# Autodesk Inventor assembly: TR2 Arm
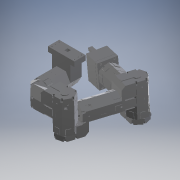
[picture p0: Inventor's stored thumbnail of the model, 180x180]
Saved by Autodesk Inventor 2017 (Build 210142000, 142)
## iProperties
Created: 2018-10-11
Part Number: TR2 Arm
Document SubType Name: Assembly
Designer: Zach
Author: Zach
## Documents named in this file (10)
- C:\Users\Dell\Documents\GitHub\tr2\Arm\Arm.iam
- C:\Users\Dell\Documents\GitHub\tr2\Arm Actuator\Arm Actuator.iam
- C:\Users\Dell\Documents\GitHub\tr2\Gripper\Gripper.iam
- C:\Users\Dell\Documents\GitHub\tr2\Arm\TARM04b.ipt
- C:\Users\Dell\Documents\GitHub\tr2\Arm\TARM09b.ipt
- C:\Users\Dell\Documents\GitHub\tr2\Arm\TARM01b.ipt
- C:\Users\Dell\Documents\GitHub\tr2\Arm\TARM02b.ipt
- C:\Users\Dell\Documents\GitHub\tr2\Arm\TARM10.ipt
- C:\Users\Dell\Documents\GitHub\tr2\Arm\TARM11.ipt
- C:\Users\Dell\Documents\GitHub\tr2\Arm\TARM12.ipt
## Components (17 placed, 9 different names)
1. TARM01b:1 — Mate:181, Mate:182, Mate:183
2. Arm Actuator:1 [sub-assembly] — Mate:181, Mate:182, Mate:183, Mate:184, Mate:185
3. Arm Actuator:2 [sub-assembly] — Mate:158, Mate:159, Mate:173, Mate:174, Mate:175
4. Arm Actuator:3 [sub-assembly] — Mate:160, Mate:161, Mate:162, Mate:176, Mate:177
5. Arm Actuator:4 [sub-assembly] — Mate:163, Mate:164, Mate:178, Mate:179, Mate:180
6. Arm Actuator:5 [sub-assembly] — Mate:165, Mate:166, Mate:167, Mate:189, Mate:206
7. Gripper:1 [sub-assembly] — Mate:189, Mate:206
8. TARM04b:1 — Mate:158, Mate:159, Mate:160, Mate:161, Mate:162, Mate:194, Mate:195, Mate:196
9. TARM04b:2 — Mate:163, Mate:164, Mate:165, Mate:166, Mate:167, Mate:197, Mate:198, Mate:199
10. TARM09b:1 — Mate:173, Mate:174, Mate:175, Mate:186, Mate:187, Mate:188, Mate:203, Mate:204, Mate:205
11. TARM09b:2 — Mate:176, Mate:177, Mate:178, Mate:179, Mate:180, Mate:200, Mate:201, Mate:202
12. TARM02b:1 — Mate:184, Mate:185, Mate:186, Mate:187, Mate:188, Mate:191, Mate:192, Mate:193
13. TARM10:1 — Mate:191, Mate:192, Mate:193
14. TARM11:1 — Mate:194, Mate:195, Mate:196
15. TARM11:2 — Mate:197, Mate:198, Mate:199
16. TARM12:1 — Mate:200, Mate:201, Mate:202
17. TARM12:2 — Mate:203, Mate:204, Mate:205
## Relationships (43: Mate 43)
- Mate:158: Arm Actuator:2 ↔ TARM04b:1
- Mate:159: Arm Actuator:2 ↔ TARM04b:1
- Mate:160: Arm Actuator:3 ↔ TARM04b:1
- Mate:161: Arm Actuator:3 ↔ TARM04b:1
- Mate:162: Arm Actuator:3 ↔ TARM04b:1
- Mate:163: Arm Actuator:4 ↔ TARM04b:2
- Mate:164: Arm Actuator:4 ↔ TARM04b:2
- Mate:165: Arm Actuator:5 ↔ TARM04b:2
- Mate:166: Arm Actuator:5 ↔ TARM04b:2
- Mate:167: Arm Actuator:5 ↔ TARM04b:2
- Mate:173: Arm Actuator:2 ↔ TARM09b:1
- Mate:174: Arm Actuator:2 ↔ TARM09b:1
- Mate:175: Arm Actuator:2 ↔ TARM09b:1
- Mate:176: Arm Actuator:3 ↔ TARM09b:2
- Mate:177: Arm Actuator:3 ↔ TARM09b:2
- Mate:178: Arm Actuator:4 ↔ TARM09b:2
- Mate:179: Arm Actuator:4 ↔ TARM09b:2
- Mate:180: Arm Actuator:4 ↔ TARM09b:2
- Mate:181: TARM01b:1 ↔ Arm Actuator:1
- Mate:182: TARM01b:1 ↔ Arm Actuator:1
- Mate:183: TARM01b:1 ↔ Arm Actuator:1
- Mate:184: Arm Actuator:1 ↔ TARM02b:1
- Mate:185: Arm Actuator:1 ↔ TARM02b:1
- Mate:186: TARM09b:1 ↔ TARM02b:1
- Mate:187: TARM09b:1 ↔ TARM02b:1
- Mate:188: TARM09b:1 ↔ TARM02b:1
- Mate:189: Arm Actuator:5 ↔ Gripper:1
- Mate:191: TARM02b:1 ↔ TARM10:1
- Mate:192: TARM02b:1 ↔ TARM10:1
- Mate:193: TARM02b:1 ↔ TARM10:1
- Mate:194: TARM04b:1 ↔ TARM11:1
- Mate:195: TARM04b:1 ↔ TARM11:1
- Mate:196: TARM04b:1 ↔ TARM11:1
- Mate:197: TARM04b:2 ↔ TARM11:2
- Mate:198: TARM04b:2 ↔ TARM11:2
- Mate:199: TARM04b:2 ↔ TARM11:2
- Mate:200: TARM09b:2 ↔ TARM12:1
- Mate:201: TARM09b:2 ↔ TARM12:1
- Mate:202: TARM09b:2 ↔ TARM12:1
- Mate:203: TARM09b:1 ↔ TARM12:2
- Mate:204: TARM09b:1 ↔ TARM12:2
- Mate:205: TARM09b:1 ↔ TARM12:2
- Mate:206: Arm Actuator:5 ↔ Gripper:1
